# Autodesk Inventor assembly: Watercooling_System
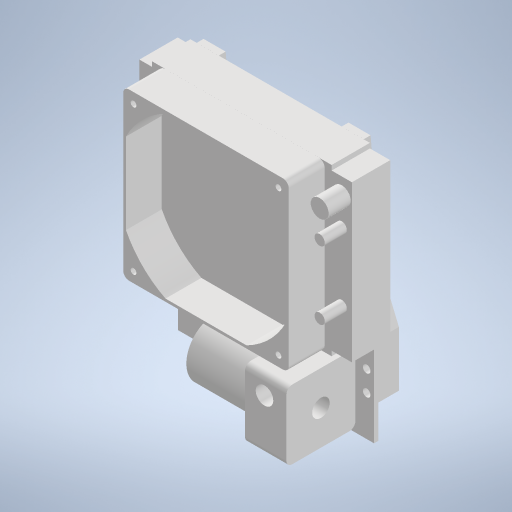
[picture p0: Inventor's stored thumbnail of the model, 512x512]
Saved by Autodesk Inventor 2023 (Build 270158000, 158)
## iProperties
Created: 2023-08-19
Part Number: Watercooling_System
Document SubType Name: Assembly
Designer: plebbb
Author: plebbb
## Documents named in this file (6)
- D:\Users\plebbb\Desktop\CNC_Project\Watercooling_System.iam
- D:\Users\plebbb\Desktop\CNC_Project\Watercooling_Rad.iam
- D:\Users\plebbb\Desktop\CNC_Project\Water_pump.ipt
- D:\Users\plebbb\Desktop\CNC_Project\Fan_side_mount.ipt
- D:\Users\plebbb\Desktop\CNC_Project\Fan_side_mount_MIR.ipt
- D:\Users\plebbb\Desktop\CNC_Project\Watercooler_Mounting_Plate.ipt
## Components (5 placed, 5 different names)
1. Watercooling_Rad:1 [sub-assembly] — Mate:3, Mate:4, Mate:6, Mate:7, Mate:8, Mate:9
2. Water_pump:1 — Mate:13, Angle:1, Mate:14, Mate:15
3. Fan_side_mount:1 — Mate:3, Mate:4, Mate:6, Flush:1, Angle:1
4. Fan_side_mount_MIR:1 — Mate:7, Mate:8, Mate:9, Mate:10, Mate:11, Mate:12
5. Watercooler_Mounting_Plate:1 — Flush:1, Mate:10, Mate:11, Mate:12, Mate:13, Mate:14, Mate:15
## Relationships (14: Mate 12, Flush 1, Angle 1)
- Mate:3: Watercooling_Rad:1 ↔ Fan_side_mount:1
- Mate:4: Watercooling_Rad:1 ↔ Fan_side_mount:1
- Mate:6: Watercooling_Rad:1 ↔ Fan_side_mount:1
- Mate:7: Watercooling_Rad:1 ↔ Fan_side_mount_MIR:1
- Mate:8: Watercooling_Rad:1 ↔ Fan_side_mount_MIR:1
- Mate:9: Watercooling_Rad:1 ↔ Fan_side_mount_MIR:1
- Flush:1: Fan_side_mount:1 ↔ Watercooler_Mounting_Plate:1
- Mate:10: Fan_side_mount_MIR:1 ↔ Watercooler_Mounting_Plate:1
- Mate:11: Fan_side_mount_MIR:1 ↔ Watercooler_Mounting_Plate:1
- Mate:12: Fan_side_mount_MIR:1 ↔ Watercooler_Mounting_Plate:1
- Mate:13: Water_pump:1 ↔ Watercooler_Mounting_Plate:1
- Angle:1 (0 deg): Water_pump:1 ↔ Fan_side_mount:1
- Mate:14: Water_pump:1 ↔ Watercooler_Mounting_Plate:1
- Mate:15: Water_pump:1 ↔ Watercooler_Mounting_Plate:1
